# Autodesk Inventor assembly: RoArm_antebrazo
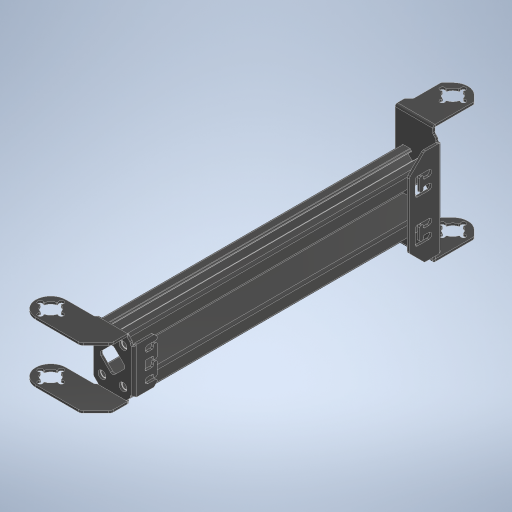
[picture p0: Inventor's stored thumbnail of the model, 512x512]
Saved by Autodesk Inventor 2024.4 (Build 284460000, 460)
## iProperties
Created: 2026-06-02
Part Number: RoArm_antebrazo
Document SubType Name: Assembly
Designer: epm01
Author: epm01
## Documents named in this file (4)
- D:\Archivos\2026-2\RoArm\inventor\RoArm_antebrazo.iam
- D:\Archivos\2026-2\RoArm\inventor\AL-SHOULDER\AL-SHOULDER\AL-SHOULDER.ipt
- D:\Archivos\2026-2\RoArm\inventor\1020铝型材200mm v2\1020铝型材200mm v2\1020铝型材200mm v2.ipt
- D:\Archivos\2026-2\RoArm\inventor\AL-ELBOW-A\AL-ELBOW-A\AL-ELBOW-A.ipt
## Components (4 placed, 3 different names)
1. AL-SHOULDER:1 — Insert:1, Flush:1, Insert:2
2. 1020铝型材200mm v2:1 — Insert:1, Flush:1, Flush:2
3. 1020铝型材200mm v2:2 — Insert:2, Flush:2, Insert:3
4. AL-ELBOW-A:1 — Insert:3
## Relationships (5: Insert 3, Flush 2)
- Insert:1: AL-SHOULDER:1 ↔ 1020铝型材200mm v2:1
- Flush:1: AL-SHOULDER:1 ↔ 1020铝型材200mm v2:1
- Insert:2: AL-SHOULDER:1 ↔ 1020铝型材200mm v2:2
- Flush:2: 1020铝型材200mm v2:1 ↔ 1020铝型材200mm v2:2
- Insert:3: 1020铝型材200mm v2:2 ↔ AL-ELBOW-A:1
